# Autodesk Inventor assembly: vrRig_v01r1_bpFull01
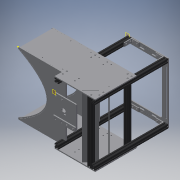
[picture p0: Inventor's stored thumbnail of the model, 180x180]
Saved by Autodesk Inventor 2016 (Build 200138000, 138)
## iProperties
Created: 2019-01-04
Part Number: vrRig_v01r1_bpFull01
Document SubType Name: Assembly
Designer: harveylab
Author: harveylab
## Documents named in this file (8)
- C:\Users\harveylab\Documents\GitHub\mouseVR\Hardware\BackProjection\vrRig_v01r1_bpFull01.iam
- C:\Users\harveylab\Documents\GitHub\mouseVR\Hardware\BackProjection\vrRig_v01r1_bpBox.iam
- C:\Users\harveylab\Documents\GitHub\mouseVR\Hardware\BackProjection\TL_XE25L18_rail.ipt
- C:\Users\harveylab\Documents\GitHub\mouseVR\Hardware\BackProjection\McM_92220A182_lowProfScrew_0p375in.ipt
- C:\Users\harveylab\Documents\GitHub\mouseVR\Hardware\BackProjection\vrRig_v01r1_base.ipt
- C:\Users\harveylab\Documents\GitHub\mouseVR\Hardware\BackProjection\McM_47065T239_cornerBracket_2in.ipt
- C:\Users\harveylab\Documents\GitHub\mouseVR\Hardware\BackProjection\vrRig_v01r1_largeMirror.ipt
- C:\Users\harveylab\Documents\GitHub\mouseVR\Hardware\BackProjection\vrRig_v01r1_smallMirror.ipt
## Components (48 placed, 7 different names)
1. vrRig_v01r1_bpBox:1 [sub-assembly] — Mate:1, Mate:2, Flush:1, Mate:3, Mate:4, Flush:2, Mate:5, Flush:3, Flush:4, Flush:5, Mate:6, Flush:6, Insert:1, Insert:2, Insert:3, Insert:4, Insert:5, Insert:6, Insert:7, Insert:8, Insert:9, Insert:10, Insert:11, Insert:12, Insert:13, Insert:14, Insert:15, Insert:16, Insert:17, Insert:18, Insert:19, Insert:20, Mate:9, Mate:10, Flush:9, Mate:11, Mate:12, Flush:10, Flush:11
2. TL_XE25L18_rail:1 — Mate:1, Mate:2, Flush:1
3. TL_XE25L18_rail:2 — Mate:3, Mate:4, Flush:2
4. TL_XE25L18_rail:3 — Mate:5, Flush:3, Flush:4
5. TL_XE25L18_rail:4 — Flush:5, Mate:6, Flush:6, Flush:7, Flush:8, Mate:8
6. McM_92220A182_lowProfScrew_0p375in:1 — Insert:1
7. McM_92220A182_lowProfScrew_0p375in:2 — Insert:2
8. McM_92220A182_lowProfScrew_0p375in:3 — Insert:3
9. McM_92220A182_lowProfScrew_0p375in:4 — Insert:4
10. McM_92220A182_lowProfScrew_0p375in:5 — Insert:8
11. McM_92220A182_lowProfScrew_0p375in:6 — Insert:7
12. McM_92220A182_lowProfScrew_0p375in:7 — Insert:6
13. McM_92220A182_lowProfScrew_0p375in:8 — Insert:5
14. McM_92220A182_lowProfScrew_0p375in:9 — Insert:16
15. McM_92220A182_lowProfScrew_0p375in:10 — Insert:11
16. McM_92220A182_lowProfScrew_0p375in:11 — Insert:10
17. McM_92220A182_lowProfScrew_0p375in:12 — Insert:9
18. McM_92220A182_lowProfScrew_0p375in:13 — Insert:12
19. McM_92220A182_lowProfScrew_0p375in:14 — Insert:13
20. McM_92220A182_lowProfScrew_0p375in:15 — Insert:14
21. McM_92220A182_lowProfScrew_0p375in:16 — Insert:15
22. McM_92220A182_lowProfScrew_0p375in:17 — Insert:17
23. McM_92220A182_lowProfScrew_0p375in:18 — Insert:19
24. McM_92220A182_lowProfScrew_0p375in:19 — Insert:18
25. McM_92220A182_lowProfScrew_0p375in:20 — Insert:20
26. vrRig_v01r1_base:1 — Flush:7, Flush:8, Mate:8, Insert:21, Insert:22, Insert:23, Insert:24, Insert:25, Insert:26, Insert:27, Insert:28
27. McM_47065T239_cornerBracket_2in:1 — Insert:25, Insert:26, Insert:33, Insert:39, Insert:40, Insert:43
28. McM_47065T239_cornerBracket_2in:2 — Insert:27, Insert:28, Insert:37, Insert:41, Insert:42, Insert:44
29. McM_47065T239_cornerBracket_2in:3 — Insert:23, Insert:24, Insert:34, Insert:35, Insert:36, Insert:38
30. McM_47065T239_cornerBracket_2in:4 — Insert:21, Insert:22, Insert:29, Insert:30, Insert:31, Insert:32
31. McM_92220A182_lowProfScrew_0p375in:21 — Insert:32
32. McM_92220A182_lowProfScrew_0p375in:22 — Insert:33
33. McM_92220A182_lowProfScrew_0p375in:23 — Insert:35
34. McM_92220A182_lowProfScrew_0p375in:24 — Insert:36
35. McM_92220A182_lowProfScrew_0p375in:25 — Insert:37
36. McM_92220A182_lowProfScrew_0p375in:26 — Insert:44
37. McM_92220A182_lowProfScrew_0p375in:27 — Insert:43
38. McM_92220A182_lowProfScrew_0p375in:28 — Insert:42
39. McM_92220A182_lowProfScrew_0p375in:29 — Insert:41
40. McM_92220A182_lowProfScrew_0p375in:30 — Insert:40
41. McM_92220A182_lowProfScrew_0p375in:31 — Insert:39
42. McM_92220A182_lowProfScrew_0p375in:32 — Insert:38
43. McM_92220A182_lowProfScrew_0p375in:33 — Insert:34
44. McM_92220A182_lowProfScrew_0p375in:34 — Insert:31
45. McM_92220A182_lowProfScrew_0p375in:35 — Insert:30
46. McM_92220A182_lowProfScrew_0p375in:36 — Insert:29
47. vrRig_v01r1_largeMirror:1 — Mate:9, Mate:10, Flush:9
48. vrRig_v01r1_smallMirror:1 — Mate:11, Mate:12, Flush:10
## Relationships (66: Insert 44, Mate 11, Flush 11)
- Mate:1: vrRig_v01r1_bpBox:1 ↔ TL_XE25L18_rail:1
- Mate:2: vrRig_v01r1_bpBox:1 ↔ TL_XE25L18_rail:1
- Flush:1: vrRig_v01r1_bpBox:1 ↔ TL_XE25L18_rail:1
- Mate:3: vrRig_v01r1_bpBox:1 ↔ TL_XE25L18_rail:2
- Mate:4: vrRig_v01r1_bpBox:1 ↔ TL_XE25L18_rail:2
- Flush:2: vrRig_v01r1_bpBox:1 ↔ TL_XE25L18_rail:2
- Mate:5: vrRig_v01r1_bpBox:1 ↔ TL_XE25L18_rail:3
- Flush:3: vrRig_v01r1_bpBox:1 ↔ TL_XE25L18_rail:3
- Flush:4: vrRig_v01r1_bpBox:1 ↔ TL_XE25L18_rail:3
- Flush:5: vrRig_v01r1_bpBox:1 ↔ TL_XE25L18_rail:4
- Mate:6: vrRig_v01r1_bpBox:1 ↔ TL_XE25L18_rail:4
- Flush:6: vrRig_v01r1_bpBox:1 ↔ TL_XE25L18_rail:4
- Insert:1: vrRig_v01r1_bpBox:1 ↔ McM_92220A182_lowProfScrew_0p375in:1
- Insert:2: vrRig_v01r1_bpBox:1 ↔ McM_92220A182_lowProfScrew_0p375in:2
- Insert:3: vrRig_v01r1_bpBox:1 ↔ McM_92220A182_lowProfScrew_0p375in:3
- Insert:4: vrRig_v01r1_bpBox:1 ↔ McM_92220A182_lowProfScrew_0p375in:4
- Insert:5: vrRig_v01r1_bpBox:1 ↔ McM_92220A182_lowProfScrew_0p375in:8
- Insert:6: vrRig_v01r1_bpBox:1 ↔ McM_92220A182_lowProfScrew_0p375in:7
- Insert:7: vrRig_v01r1_bpBox:1 ↔ McM_92220A182_lowProfScrew_0p375in:6
- Insert:8: vrRig_v01r1_bpBox:1 ↔ McM_92220A182_lowProfScrew_0p375in:5
- Insert:9: vrRig_v01r1_bpBox:1 ↔ McM_92220A182_lowProfScrew_0p375in:12
- Insert:10: vrRig_v01r1_bpBox:1 ↔ McM_92220A182_lowProfScrew_0p375in:11
- Insert:11: vrRig_v01r1_bpBox:1 ↔ McM_92220A182_lowProfScrew_0p375in:10
- Insert:12: vrRig_v01r1_bpBox:1 ↔ McM_92220A182_lowProfScrew_0p375in:13
- Insert:13: vrRig_v01r1_bpBox:1 ↔ McM_92220A182_lowProfScrew_0p375in:14
- Insert:14: vrRig_v01r1_bpBox:1 ↔ McM_92220A182_lowProfScrew_0p375in:15
- Insert:15: vrRig_v01r1_bpBox:1 ↔ McM_92220A182_lowProfScrew_0p375in:16
- Insert:16: vrRig_v01r1_bpBox:1 ↔ McM_92220A182_lowProfScrew_0p375in:9
- Insert:17: vrRig_v01r1_bpBox:1 ↔ McM_92220A182_lowProfScrew_0p375in:17
- Insert:18: vrRig_v01r1_bpBox:1 ↔ McM_92220A182_lowProfScrew_0p375in:19
- Insert:19: vrRig_v01r1_bpBox:1 ↔ McM_92220A182_lowProfScrew_0p375in:18
- Insert:20: vrRig_v01r1_bpBox:1 ↔ McM_92220A182_lowProfScrew_0p375in:20
- Flush:7: TL_XE25L18_rail:4 ↔ vrRig_v01r1_base:1
- Flush:8: TL_XE25L18_rail:4 ↔ vrRig_v01r1_base:1
- Mate:8: TL_XE25L18_rail:4 ↔ vrRig_v01r1_base:1
- Insert:21: vrRig_v01r1_base:1 ↔ McM_47065T239_cornerBracket_2in:4
- Insert:22: vrRig_v01r1_base:1 ↔ McM_47065T239_cornerBracket_2in:4
- Insert:23: vrRig_v01r1_base:1 ↔ McM_47065T239_cornerBracket_2in:3
- Insert:24: vrRig_v01r1_base:1 ↔ McM_47065T239_cornerBracket_2in:3
- Insert:25: vrRig_v01r1_base:1 ↔ McM_47065T239_cornerBracket_2in:1
- Insert:26: vrRig_v01r1_base:1 ↔ McM_47065T239_cornerBracket_2in:1
- Insert:27: vrRig_v01r1_base:1 ↔ McM_47065T239_cornerBracket_2in:2
- Insert:28: vrRig_v01r1_base:1 ↔ McM_47065T239_cornerBracket_2in:2
- Insert:29: McM_47065T239_cornerBracket_2in:4 ↔ McM_92220A182_lowProfScrew_0p375in:36
- Insert:30: McM_47065T239_cornerBracket_2in:4 ↔ McM_92220A182_lowProfScrew_0p375in:35
- Insert:31: McM_47065T239_cornerBracket_2in:4 ↔ McM_92220A182_lowProfScrew_0p375in:34
- Insert:32: McM_47065T239_cornerBracket_2in:4 ↔ McM_92220A182_lowProfScrew_0p375in:21
- Insert:33: McM_47065T239_cornerBracket_2in:1 ↔ McM_92220A182_lowProfScrew_0p375in:22
- Insert:34: McM_47065T239_cornerBracket_2in:3 ↔ McM_92220A182_lowProfScrew_0p375in:33
- Insert:35: McM_47065T239_cornerBracket_2in:3 ↔ McM_92220A182_lowProfScrew_0p375in:23
- Insert:36: McM_47065T239_cornerBracket_2in:3 ↔ McM_92220A182_lowProfScrew_0p375in:24
- Insert:37: McM_47065T239_cornerBracket_2in:2 ↔ McM_92220A182_lowProfScrew_0p375in:25
- Insert:38: McM_47065T239_cornerBracket_2in:3 ↔ McM_92220A182_lowProfScrew_0p375in:32
- Insert:39: McM_47065T239_cornerBracket_2in:1 ↔ McM_92220A182_lowProfScrew_0p375in:31
- Insert:40: McM_47065T239_cornerBracket_2in:1 ↔ McM_92220A182_lowProfScrew_0p375in:30
- Insert:41: McM_47065T239_cornerBracket_2in:2 ↔ McM_92220A182_lowProfScrew_0p375in:29
- Insert:42: McM_47065T239_cornerBracket_2in:2 ↔ McM_92220A182_lowProfScrew_0p375in:28
- Insert:43: McM_47065T239_cornerBracket_2in:1 ↔ McM_92220A182_lowProfScrew_0p375in:27
- Insert:44: McM_47065T239_cornerBracket_2in:2 ↔ McM_92220A182_lowProfScrew_0p375in:26
- Mate:9: vrRig_v01r1_bpBox:1 ↔ vrRig_v01r1_largeMirror:1
- Mate:10: vrRig_v01r1_bpBox:1 ↔ vrRig_v01r1_largeMirror:1
- Flush:9: vrRig_v01r1_bpBox:1 ↔ vrRig_v01r1_largeMirror:1
- Mate:11: vrRig_v01r1_bpBox:1 ↔ vrRig_v01r1_smallMirror:1
- Mate:12: vrRig_v01r1_bpBox:1 ↔ vrRig_v01r1_smallMirror:1
- Flush:10: vrRig_v01r1_bpBox:1 ↔ vrRig_v01r1_smallMirror:1
- Flush:11: vrRig_v01r1_bpBox:1
